# Autodesk Inventor assembly: 2016-01-31-LiftTiltAssembly
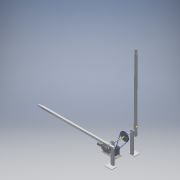
[picture p0: Inventor's stored thumbnail of the model, 180x180]
Saved by Autodesk Inventor 2016 SP1 (Build 200210100, 210)
## iProperties
Created: 2016-02-01
Part Number: 2016-01-31-LiftTiltAssembly
Document SubType Name: Assembly
Designer: steele
Mass: 1180.85 g
Surface Area: 3067.44 cm^2
Volume: 579.525 cm^3
Density: 2.03761 g/cm^3
Author: steele
## Documents named in this file (10)
- C:\snobotics\CAD-Development\robSteele\SnoBotics2016\2016-01-31-Lift\2016-01-31-LiftTiltAssembly.iam
- C:\snobotics\CAD-Development\robSteele\SnoBotics2016\AM Parts\rsSnowBlowerMount.ipt
- C:\snobotics\CAD-Development\robSteele\SnoBotics2016\AM Parts\AM-2235-snow-blower_MIR.iam
- C:\snobotics\CAD-Development\robSteele\SnoBotics2016\2016-01-31-Lift\2016-01-31-LiftTiltAssembly\Design Accelerator\Chain Drive1.iam
- C:\snobotics\CAD-Development\robSteele\SnoBotics2016\2016-01-31-Lift\2016-01-31-LiftTiltAssembly\Design Accelerator\Chain Drive2.iam
- C:\snobotics\CAD-Development\robSteele\SnoBotics2016\2016-01-31-Lift\MiddlePostForLift.ipt
- C:\snobotics\CAD-Development\robSteele\SnoBotics2016\2016-01-31-Lift\dualLiftAxel.ipt
- C:\snobotics\CAD-Development\robSteele\SnoBotics2016\2016-01-31-Lift\TelescopingArmSpringDriven.iam
- C:\snobotics\CAD-Development\robSteele\SnoBotics2016\2016-01-31-Lift\TelescopingArmSpringDriven_MIR1.iam
- C:\snobotics\CAD-Development\robSteele\SnoBotics2016\2016-01-31-Lift\RearPostForLiftWith2Posts.ipt
## Components (9 placed, 8 different names)
1. rsSnowBlowerMount:1 — Flush:1, Mate:1, Flush:2, Insert:1, Flush:3, Flush:4
2. AM-2235-snow-blower_MIR:1 [sub-assembly] — Insert:1
3. MiddlePostForLift:1 — Flush:1, Mate:1, Flush:2, Mate:2
4. Chain Drive:1 [sub-assembly]
5. RearPostForLiftWith2Posts:1 — Flush:3, Flush:4, Mate:2, Insert:4
6. Chain Drive:2 [sub-assembly]
7. dualLiftAxel:1 — Insert:2, Insert:3
8. TelescopingArmSpringDriven:1 [sub-assembly] — Insert:2, Insert:4
9. TelescopingArmSpringDriven_MIR1:1 [sub-assembly] — Insert:3
## Relationships (10: Flush 4, Insert 4, Mate 2)
- Flush:1: rsSnowBlowerMount:1 ↔ MiddlePostForLift:1
- Mate:1 (6.35 mm): rsSnowBlowerMount:1 ↔ MiddlePostForLift:1
- Flush:2: rsSnowBlowerMount:1 ↔ MiddlePostForLift:1
- Insert:1: rsSnowBlowerMount:1 ↔ AM-2235-snow-blower_MIR:1
- Flush:3: rsSnowBlowerMount:1 ↔ RearPostForLiftWith2Posts:1
- Flush:4: rsSnowBlowerMount:1 ↔ RearPostForLiftWith2Posts:1
- Mate:2 (6.35 mm): MiddlePostForLift:1 ↔ RearPostForLiftWith2Posts:1
- Insert:2: dualLiftAxel:1 ↔ TelescopingArmSpringDriven:1
- Insert:3: dualLiftAxel:1 ↔ TelescopingArmSpringDriven_MIR1:1
- Insert:4 (55.5752 mm): RearPostForLiftWith2Posts:1 ↔ TelescopingArmSpringDriven:1
